# Autodesk Inventor assembly: assy_parkinglot_rear_left
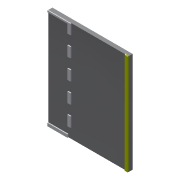
[picture p0: Inventor's stored thumbnail of the model, 180x180]
Saved by Autodesk Inventor 2018 (Build 220112000, 112)
## iProperties
Created: 2017-11-13
Part Number: assy_parkinglot_rear_left
Document SubType Name: Assembly
Designer: Platform
Author: Platform
## Documents named in this file (6)
- C:\Users\Platform\Desktop\autorace_track\track_model\autorace_rbizchallenge2017\assembled\assy_parkinglot_rear_left.iam
- C:\Users\Platform\Desktop\autorace_track\track_model\autorace_rbizchallenge2017\parts\ipt\upper_plate_parking1 v1.ipt
- C:\Users\Platform\Desktop\autorace_track\track_model\autorace_rbizchallenge2017\parts\ipt\straight_line.ipt
- C:\Users\Platform\Desktop\autorace_track\track_model\autorace_rbizchallenge2017\parts\ipt\straight_line_dotted_parkinglot.ipt
- C:\Users\Platform\Desktop\autorace_track\track_model\autorace_rbizchallenge2017\parts\ipt\line_edge_parkinglot_1_1.ipt
- C:\Users\Platform\Desktop\autorace_track\track_model\autorace_rbizchallenge2017\parts\ipt\line_edge_parkinglot_1_2.ipt
## Components (9 placed, 5 different names)
1. upper_plate_parking1 v1:1 — Mate:2, Flush:1, Flush:2, Mate:3, Mate:5, Mate:6, Mate:7, Mate:11, Flush:7, Mate:12, Flush:9, Flush:10, Flush:11
2. straight_line:1
3. straight_line_dotted_parkinglot:1 — Mate:2, Flush:1, Flush:2, Flush:3, Mate:4
4. straight_line_dotted_parkinglot:2 — Mate:3, Flush:3, Mate:4, Mate:8, Flush:4
5. straight_line_dotted_parkinglot:3 — Mate:5, Mate:8, Flush:4, Mate:9, Flush:5
6. straight_line_dotted_parkinglot:4 — Mate:6, Mate:9, Flush:5, Mate:10, Flush:6
7. straight_line_dotted_parkinglot:5 — Mate:7, Mate:10, Flush:6
8. line_edge_parkinglot_1_1:1 — Mate:11, Flush:7, Flush:11
9. line_edge_parkinglot_1_2:1 — Mate:12, Flush:9, Flush:10
## Relationships (22: Mate 12, Flush 10)
- [Mate]: upper_plate_parking1 v1:1 ↔ straight_line:1
- Mate:2: upper_plate_parking1 v1:1 ↔ straight_line_dotted_parkinglot:1
- Flush:1: upper_plate_parking1 v1:1 ↔ straight_line_dotted_parkinglot:1
- Flush:2 (100 mm): upper_plate_parking1 v1:1 ↔ straight_line_dotted_parkinglot:1
- Mate:3: upper_plate_parking1 v1:1 ↔ straight_line_dotted_parkinglot:2
- Flush:3: straight_line_dotted_parkinglot:1 ↔ straight_line_dotted_parkinglot:2
- Mate:4 (50 mm): straight_line_dotted_parkinglot:1 ↔ straight_line_dotted_parkinglot:2
- Mate:5: upper_plate_parking1 v1:1 ↔ straight_line_dotted_parkinglot:3
- Mate:6: upper_plate_parking1 v1:1 ↔ straight_line_dotted_parkinglot:4
- Mate:7: upper_plate_parking1 v1:1 ↔ straight_line_dotted_parkinglot:5
- Mate:8 (50 mm): straight_line_dotted_parkinglot:2 ↔ straight_line_dotted_parkinglot:3
- Flush:4: straight_line_dotted_parkinglot:2 ↔ straight_line_dotted_parkinglot:3
- Mate:9 (50 mm): straight_line_dotted_parkinglot:3 ↔ straight_line_dotted_parkinglot:4
- Flush:5: straight_line_dotted_parkinglot:3 ↔ straight_line_dotted_parkinglot:4
- Mate:10 (50 mm): straight_line_dotted_parkinglot:4 ↔ straight_line_dotted_parkinglot:5
- Flush:6: straight_line_dotted_parkinglot:4 ↔ straight_line_dotted_parkinglot:5
- Mate:11: upper_plate_parking1 v1:1 ↔ line_edge_parkinglot_1_1:1
- Flush:7: upper_plate_parking1 v1:1 ↔ line_edge_parkinglot_1_1:1
- Mate:12: upper_plate_parking1 v1:1 ↔ line_edge_parkinglot_1_2:1
- Flush:9: upper_plate_parking1 v1:1 ↔ line_edge_parkinglot_1_2:1
- Flush:10: upper_plate_parking1 v1:1 ↔ line_edge_parkinglot_1_2:1
- Flush:11: upper_plate_parking1 v1:1 ↔ line_edge_parkinglot_1_1:1
